# Autodesk Inventor assembly: Chassis_Base
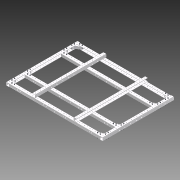
[picture p0: Inventor's stored thumbnail of the model, 180x180]
Saved by Autodesk Inventor 2012 SP1 (Build 160190100, 190)
## iProperties
Category: Chassis
Company: Autodesk Inc.
Created: 2009-11-26
Part Number: Chassis_Base
Document SubType Name: Assembly
Designer: Autodesk Inc.
Catalog Web Link: http://andymark.biz/am-0453.html
Description: C-base chassis
Vendor: Andy Mark
Mass: 5433.99 g
Surface Area: 12265.2 cm^2
Volume: 2015.03 cm^3
Density: 2.69673 g/cm^3
Author: Autodesk Inc.
## Documents named in this file (7)
- K:\MHS\Technology\Holliday B\Group Projects\Robotics\CAD Team\CAD Team 2013\Chassis\Full Chassis\Chassis_Base.iam
- K:\MHS\Technology\Holliday B\Group Projects\Robotics\CAD Team\Ian CAD\Robotics\Chasis\Chassis_Channel_AndyMark_am-0202.ipt
- K:\MHS\Technology\Holliday B\Group Projects\Robotics\CAD Team\Ian CAD\Robotics\Chasis\Chassis_CornerConnect_AndyMark_am-0212.ipt
- K:\MHS\Technology\Holliday B\Group Projects\Robotics\CAD Team\Ian CAD\Robotics\Chasis\Chassis_Channel_26_AndyMark_am-0202.ipt
- K:\MHS\Technology\Holliday B\Group Projects\Robotics\CAD Team\Ian CAD\Robotics\Chasis\SHCS_NylockNut_Corner.iam
- K:\MHS\Technology\Holliday B\Group Projects\Robotics\CAD Team\2012 Robot\Chassis\Frame\Chassis_Channel_10_AndyMark_am-0202.ipt
- K:\MHS\Technology\Holliday B\Group Projects\Robotics\CAD Team\Ian CAD\Robotics\Chasis\Chassis_Channel_AndyMark_am-0202_CPY.ipt
## Components (36 placed, 6 different names)
1. Chassis_Channel_AndyMark_am-0202:1 — Mate:1, Flush:1, Insert:2, Mate:2, Flush:2, Mate:19, Mate:20, Insert:37, Insert:38, Insert:74, Insert:86, Insert:87, Insert:151, Insert:153
2. Chassis_Channel_AndyMark_am-0202:2 — Flush:3, Insert:7, Mate:24, Mate:25, Insert:43, Insert:44, Insert:49, Insert:50, Mate:32, Insert:121
3. Chassis_CornerConnect_AndyMark_am-0212:1 — Insert:2, Insert:95
4. Chassis_CornerConnect_AndyMark_am-0212:2 — Insert:74, Insert:104
5. Chassis_CornerConnect_AndyMark_am-0212:3 — Insert:7, Insert:122
6. Chassis_CornerConnect_AndyMark_am-0212:4 — Insert:121, Insert:123
7. Chassis_CornerConnect_AndyMark_am-0212:5 — Insert:115, Insert:116, Insert:138, Insert:139
8. Chassis_CornerConnect_AndyMark_am-0212:8 — Insert:90, Insert:91, Insert:118, Insert:119
9. Chassis_Channel_26_AndyMark_am-0202:1 — Mate:1, Flush:1, Flush:3, Insert:95, Insert:113, Insert:114, Insert:115, Insert:116, Mate:32, Insert:123, Insert:126, Insert:127, Insert:128, Insert:129, Insert:142, Insert:143, Insert:162, Insert:163
10. Chassis_Channel_26_AndyMark_am-0202:2 — Mate:2, Flush:2, Insert:104, Insert:111, Insert:117, Insert:118, Insert:119, Insert:122, Insert:124, Insert:125, Insert:130, Insert:131, Insert:146, Insert:147, Flush:36, Mate:36, Flush:37, Mate:37, Insert:164, Insert:165
11. SHCS_NylockNut_Corner:5 [sub-assembly] — Insert:43, Insert:44
12. SHCS_NylockNut_Corner:6 [sub-assembly] — Insert:49, Insert:50
13. SHCS_NylockNut_Corner:2 [sub-assembly] — Insert:37, Insert:38
14. SHCS_NylockNut_Corner:9 [sub-assembly] — Insert:140, Insert:141
15. SHCS_NylockNut_Corner:10 [sub-assembly] — Insert:101
16. SHCS_NylockNut_Corner:11 [sub-assembly] — Insert:86, Insert:87
17. Chassis_Channel_10_AndyMark_am-0202:1 — Insert:138, Insert:139, Insert:140, Insert:141, Insert:150
18. Chassis_Channel_10_AndyMark_am-0202:2 — Insert:90, Insert:91, Insert:101, Insert:152
19. SHCS_NylockNut_Corner:12 [sub-assembly] — Insert:111, Insert:117
20. SHCS_NylockNut_Corner:13 [sub-assembly] — Insert:113, Insert:114
21. SHCS_NylockNut_Corner:14 [sub-assembly] — Insert:126, Insert:127
22. SHCS_NylockNut_Corner:15 [sub-assembly] — Insert:124, Insert:125
23. SHCS_NylockNut_Corner:16 [sub-assembly] — Insert:128, Insert:129
24. SHCS_NylockNut_Corner:17 [sub-assembly] — Insert:130, Insert:131
25. Chassis_Channel_10_AndyMark_am-0202:3 — Insert:148, Insert:149, Flush:38, Insert:166, Insert:167
26. Chassis_Channel_10_AndyMark_am-0202:4 — Insert:144, Insert:145
27. Chassis_CornerConnect_AndyMark_am-0212:9 — Insert:146, Insert:147, Insert:148, Insert:149
28. Chassis_CornerConnect_AndyMark_am-0212:10 — Insert:142, Insert:143, Insert:144, Insert:145
29. Chassis_Channel_26_AndyMark_am-0202:3 — Insert:152, Insert:153
30. Chassis_Channel_26_AndyMark_am-0202:4 — Insert:150, Insert:151, Mate:35
31. Chassis_Channel_AndyMark_am-0202_CPY:1 — Mate:33, Mate:34, Mate:36, Flush:37, Flush:38, Insert:160, Insert:161
32. Chassis_Channel_AndyMark_am-0202_CPY:2 — Mate:35, Flush:36, Mate:37
33. SHCS_NylockNut_Corner:18 [sub-assembly] — Insert:160, Insert:161
34. SHCS_NylockNut_Corner:19 [sub-assembly] — Insert:162, Insert:163
35. SHCS_NylockNut_Corner:20 [sub-assembly] — Insert:164, Insert:165
36. SHCS_NylockNut_Corner:21 [sub-assembly] — Insert:166, Insert:167
## Relationships (77: Insert 59, Mate 12, Flush 6)
- Mate:1: Chassis_Channel_AndyMark_am-0202:1 ↔ Chassis_Channel_26_AndyMark_am-0202:1
- Flush:1: Chassis_Channel_AndyMark_am-0202:1 ↔ Chassis_Channel_26_AndyMark_am-0202:1
- Insert:2: Chassis_Channel_AndyMark_am-0202:1 ↔ Chassis_CornerConnect_AndyMark_am-0212:1
- Mate:2: Chassis_Channel_AndyMark_am-0202:1 ↔ Chassis_Channel_26_AndyMark_am-0202:2
- Flush:2: Chassis_Channel_AndyMark_am-0202:1 ↔ Chassis_Channel_26_AndyMark_am-0202:2
- Flush:3: Chassis_Channel_AndyMark_am-0202:2 ↔ Chassis_Channel_26_AndyMark_am-0202:1
- Insert:7: Chassis_Channel_AndyMark_am-0202:2 ↔ Chassis_CornerConnect_AndyMark_am-0212:3
- Mate:19: Chassis_Channel_AndyMark_am-0202:1
- Mate:20: Chassis_Channel_AndyMark_am-0202:1
- Mate:24: Chassis_Channel_AndyMark_am-0202:2
- Mate:25: Chassis_Channel_AndyMark_am-0202:2
- Insert:37: Chassis_Channel_AndyMark_am-0202:1 ↔ SHCS_NylockNut_Corner:2
- Insert:38: Chassis_Channel_AndyMark_am-0202:1 ↔ SHCS_NylockNut_Corner:2
- Insert:43: Chassis_Channel_AndyMark_am-0202:2 ↔ SHCS_NylockNut_Corner:5
- Insert:44: Chassis_Channel_AndyMark_am-0202:2 ↔ SHCS_NylockNut_Corner:5
- Insert:49: Chassis_Channel_AndyMark_am-0202:2 ↔ SHCS_NylockNut_Corner:6
- Insert:50: Chassis_Channel_AndyMark_am-0202:2 ↔ SHCS_NylockNut_Corner:6
- Insert:74: Chassis_Channel_AndyMark_am-0202:1 ↔ Chassis_CornerConnect_AndyMark_am-0212:2
- Insert:86: Chassis_Channel_AndyMark_am-0202:1 ↔ SHCS_NylockNut_Corner:11
- Insert:87: Chassis_Channel_AndyMark_am-0202:1 ↔ SHCS_NylockNut_Corner:11
- Insert:90: Chassis_CornerConnect_AndyMark_am-0212:8 ↔ Chassis_Channel_10_AndyMark_am-0202:2
- Insert:91: Chassis_CornerConnect_AndyMark_am-0212:8 ↔ Chassis_Channel_10_AndyMark_am-0202:2
- Insert:95: Chassis_CornerConnect_AndyMark_am-0212:1 ↔ Chassis_Channel_26_AndyMark_am-0202:1
- Insert:101: SHCS_NylockNut_Corner:10 ↔ Chassis_Channel_10_AndyMark_am-0202:2
- Insert:104: Chassis_CornerConnect_AndyMark_am-0212:2 ↔ Chassis_Channel_26_AndyMark_am-0202:2
- Insert:111: Chassis_Channel_26_AndyMark_am-0202:2 ↔ SHCS_NylockNut_Corner:12
- Insert:113: Chassis_Channel_26_AndyMark_am-0202:1 ↔ SHCS_NylockNut_Corner:13
- Insert:114: Chassis_Channel_26_AndyMark_am-0202:1 ↔ SHCS_NylockNut_Corner:13
- Insert:115: Chassis_CornerConnect_AndyMark_am-0212:5 ↔ Chassis_Channel_26_AndyMark_am-0202:1
- Insert:116: Chassis_CornerConnect_AndyMark_am-0212:5 ↔ Chassis_Channel_26_AndyMark_am-0202:1
- Insert:117: Chassis_Channel_26_AndyMark_am-0202:2 ↔ SHCS_NylockNut_Corner:12
- Insert:118: Chassis_CornerConnect_AndyMark_am-0212:8 ↔ Chassis_Channel_26_AndyMark_am-0202:2
- Insert:119: Chassis_CornerConnect_AndyMark_am-0212:8 ↔ Chassis_Channel_26_AndyMark_am-0202:2
- Mate:32: Chassis_Channel_AndyMark_am-0202:2 ↔ Chassis_Channel_26_AndyMark_am-0202:1
- Insert:121: Chassis_Channel_AndyMark_am-0202:2 ↔ Chassis_CornerConnect_AndyMark_am-0212:4
- Insert:122: Chassis_CornerConnect_AndyMark_am-0212:3 ↔ Chassis_Channel_26_AndyMark_am-0202:2
- Insert:123: Chassis_CornerConnect_AndyMark_am-0212:4 ↔ Chassis_Channel_26_AndyMark_am-0202:1
- Insert:124: Chassis_Channel_26_AndyMark_am-0202:2 ↔ SHCS_NylockNut_Corner:15
- Insert:125: Chassis_Channel_26_AndyMark_am-0202:2 ↔ SHCS_NylockNut_Corner:15
- Insert:126: Chassis_Channel_26_AndyMark_am-0202:1 ↔ SHCS_NylockNut_Corner:14
- Insert:127: Chassis_Channel_26_AndyMark_am-0202:1 ↔ SHCS_NylockNut_Corner:14
- Insert:128: Chassis_Channel_26_AndyMark_am-0202:1 ↔ SHCS_NylockNut_Corner:16
- Insert:129: Chassis_Channel_26_AndyMark_am-0202:1 ↔ SHCS_NylockNut_Corner:16
- Insert:130: Chassis_Channel_26_AndyMark_am-0202:2 ↔ SHCS_NylockNut_Corner:17
- Insert:131: Chassis_Channel_26_AndyMark_am-0202:2 ↔ SHCS_NylockNut_Corner:17
- Insert:138: Chassis_CornerConnect_AndyMark_am-0212:5 ↔ Chassis_Channel_10_AndyMark_am-0202:1
- Insert:139: Chassis_CornerConnect_AndyMark_am-0212:5 ↔ Chassis_Channel_10_AndyMark_am-0202:1
- Insert:140: SHCS_NylockNut_Corner:9 ↔ Chassis_Channel_10_AndyMark_am-0202:1
- Insert:141: SHCS_NylockNut_Corner:9 ↔ Chassis_Channel_10_AndyMark_am-0202:1
- Insert:142: Chassis_Channel_26_AndyMark_am-0202:1 ↔ Chassis_CornerConnect_AndyMark_am-0212:10
- Insert:143: Chassis_Channel_26_AndyMark_am-0202:1 ↔ Chassis_CornerConnect_AndyMark_am-0212:10
- Insert:144: Chassis_Channel_10_AndyMark_am-0202:4 ↔ Chassis_CornerConnect_AndyMark_am-0212:10
- Insert:145: Chassis_Channel_10_AndyMark_am-0202:4 ↔ Chassis_CornerConnect_AndyMark_am-0212:10
- Insert:146: Chassis_Channel_26_AndyMark_am-0202:2 ↔ Chassis_CornerConnect_AndyMark_am-0212:9
- Insert:147: Chassis_Channel_26_AndyMark_am-0202:2 ↔ Chassis_CornerConnect_AndyMark_am-0212:9
- Insert:148: Chassis_Channel_10_AndyMark_am-0202:3 ↔ Chassis_CornerConnect_AndyMark_am-0212:9
- Insert:149: Chassis_Channel_10_AndyMark_am-0202:3 ↔ Chassis_CornerConnect_AndyMark_am-0212:9
- Insert:150: Chassis_Channel_10_AndyMark_am-0202:1 ↔ Chassis_Channel_26_AndyMark_am-0202:4
- Insert:151: Chassis_Channel_AndyMark_am-0202:1 ↔ Chassis_Channel_26_AndyMark_am-0202:4
- Insert:152: Chassis_Channel_10_AndyMark_am-0202:2 ↔ Chassis_Channel_26_AndyMark_am-0202:3
- Insert:153: Chassis_Channel_AndyMark_am-0202:1 ↔ Chassis_Channel_26_AndyMark_am-0202:3
- Mate:33: Chassis_Channel_AndyMark_am-0202_CPY:1
- Mate:34: Chassis_Channel_AndyMark_am-0202_CPY:1
- Mate:35: Chassis_Channel_26_AndyMark_am-0202:4 ↔ Chassis_Channel_AndyMark_am-0202_CPY:2
- Flush:36: Chassis_Channel_26_AndyMark_am-0202:2 ↔ Chassis_Channel_AndyMark_am-0202_CPY:2
- Mate:36: Chassis_Channel_26_AndyMark_am-0202:2 ↔ Chassis_Channel_AndyMark_am-0202_CPY:1
- Flush:37: Chassis_Channel_26_AndyMark_am-0202:2 ↔ Chassis_Channel_AndyMark_am-0202_CPY:1
- Flush:38: Chassis_Channel_10_AndyMark_am-0202:3 ↔ Chassis_Channel_AndyMark_am-0202_CPY:1
- Mate:37: Chassis_Channel_26_AndyMark_am-0202:2 ↔ Chassis_Channel_AndyMark_am-0202_CPY:2
- Insert:160: Chassis_Channel_AndyMark_am-0202_CPY:1 ↔ SHCS_NylockNut_Corner:18
- Insert:161: Chassis_Channel_AndyMark_am-0202_CPY:1 ↔ SHCS_NylockNut_Corner:18
- Insert:162: Chassis_Channel_26_AndyMark_am-0202:1 ↔ SHCS_NylockNut_Corner:19
- Insert:163: Chassis_Channel_26_AndyMark_am-0202:1 ↔ SHCS_NylockNut_Corner:19
- Insert:164: Chassis_Channel_26_AndyMark_am-0202:2 ↔ SHCS_NylockNut_Corner:20
- Insert:165: Chassis_Channel_26_AndyMark_am-0202:2 ↔ SHCS_NylockNut_Corner:20
- Insert:166: Chassis_Channel_10_AndyMark_am-0202:3 ↔ SHCS_NylockNut_Corner:21
- Insert:167: Chassis_Channel_10_AndyMark_am-0202:3 ↔ SHCS_NylockNut_Corner:21
